# Autodesk Inventor assembly: MontagemSemPosicionamento
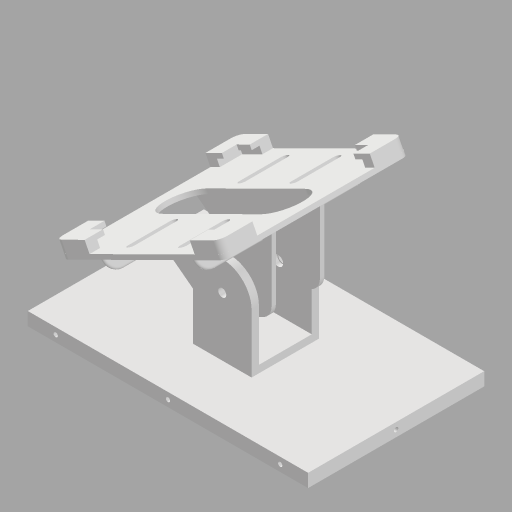
[picture p0: Inventor's stored thumbnail of the model, 512x512]
Saved by Autodesk Inventor 2023.2 (Build 272271030, 271C)
## iProperties
Created: 2024-06-18
Part Number: MontagemSemPosicionamento
Document SubType Name: Assembly
Designer: VICTOR
Author: VICTOR
## Documents named in this file (5)
- C:\Users\VICTOR\OneDrive\Área de Trabalho\TCC_Final\modelagem3D\modelosCAD\MontagemSemPosicionamento.iam
- C:\Users\VICTOR\OneDrive\Área de Trabalho\TCC_Final\modelagem3D\modelosCAD\Part1_Fixo_30_60_largo_7mm.ipt
- C:\Users\VICTOR\OneDrive\Área de Trabalho\TCC_Final\modelagem3D\modelosCAD\Apoio_Fixo_4640.ipt
- C:\Users\VICTOR\OneDrive\Área de Trabalho\TCC_Final\modelagem3D\modelosCAD\Lateral1-2.ipt
- C:\Users\VICTOR\OneDrive\Área de Trabalho\TCC_Final\modelagem3D\modelosCAD\PresasPlaca_4.ipt
## Components (7 placed, 4 different names)
1. Part1_Fixo_30_60_largo_7mm:1 — Rigid:1, Rigid:3, Rigid:4, Rigid:5, Rigid:6
2. Lateral1-2:1 — Rigid:2
3. Apoio_Fixo_4640:1 — Rigid:1, Rigid:2
4. PresasPlaca_4:1 — Rigid:3
5. PresasPlaca_4:2 — Rigid:4
6. PresasPlaca_4:3 — Rigid:5
7. PresasPlaca_4:4 — Rigid:6
## Relationships (6: WeldJoint 6)
- Rigid:1 [WeldJoint]: Part1_Fixo_30_60_largo_7mm:1 ↔ Apoio_Fixo_4640:1
- Rigid:2 [WeldJoint]: Lateral1-2:1 ↔ Apoio_Fixo_4640:1
- Rigid:3 [WeldJoint]: Part1_Fixo_30_60_largo_7mm:1 ↔ PresasPlaca_4:1
- Rigid:4 [WeldJoint]: Part1_Fixo_30_60_largo_7mm:1 ↔ PresasPlaca_4:2
- Rigid:5 [WeldJoint]: Part1_Fixo_30_60_largo_7mm:1 ↔ PresasPlaca_4:3
- Rigid:6 [WeldJoint]: Part1_Fixo_30_60_largo_7mm:1 ↔ PresasPlaca_4:4
